# Autodesk Inventor assembly: GI - 100
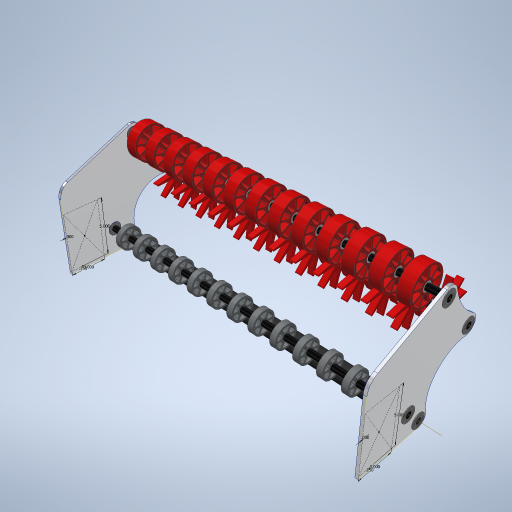
[picture p0: Inventor's stored thumbnail of the model, 512x512]
Saved by Autodesk Inventor 2023.4 (Build 274418000, 418)
## iProperties
Created: 2025-01-18
Part Number: GI - 100
Document SubType Name: Assembly
Designer: mavericks
Author: mavericks
## Documents named in this file (8)
- C:\Users\mavericks\Documents\GitHub\2025-ReefScape---CAD\ground intake\GI - 100.iam
- C:\Users\mavericks\Documents\GitHub\2025-ReefScape---CAD\ground intake\GI - 001.ipt
- C:\Users\mavericks\Documents\GitHub\2025-ReefScape---CAD\COMMON PARTS\BEARINGS\13_75mm_1_2_ThunderHex_ID_x_1_125_OD_x_0_313_WD_Flanged_Bearing_217-4006_MIR.ipt
- C:\Users\mavericks\Documents\GitHub\2025-ReefScape---CAD\ground intake\GI - 002.ipt
- C:\Users\mavericks\Documents\GitHub\2025-ReefScape---CAD\COMMON PARTS\WHEELS\am-0619a .425 Hex Entrapption Star REV2.ipt
- C:\Users\mavericks\Documents\GitHub\2025-ReefScape---CAD\COMMON PARTS\WHEELS\am-3946 3IN 375Hex Compliant Wheel REV 3.ipt
- C:\Users\mavericks\Documents\GitHub\2025-ReefScape---CAD\COMMON PARTS\WHEELS\2_OD_Straight_Flex_Wheel_217-6354.ipt
- C:\Users\mavericks\Documents\GitHub\2025-ReefScape---CAD\ground intake\GI - 200.iam
## Components (53 placed, 7 different names)
1. GI - 001:1 — Insert:1, Insert:2, Insert:3, Insert:4, Mate:2, Mate:4, Mate:6
2. 13_75mm_1_2_ThunderHex_ID_x_1_125_OD_x_0_313_WD_Flanged_Bearing_217-4006_MIR:1 — Insert:2, Insert:11, Mate:1
3. 13_75mm_1_2_ThunderHex_ID_x_1_125_OD_x_0_313_WD_Flanged_Bearing_217-4006_MIR:2 — Insert:1, Insert:12, Mate:3
4. 13_75mm_1_2_ThunderHex_ID_x_1_125_OD_x_0_313_WD_Flanged_Bearing_217-4006_MIR:3 — Insert:4, Insert:17
5. 13_75mm_1_2_ThunderHex_ID_x_1_125_OD_x_0_313_WD_Flanged_Bearing_217-4006_MIR:4 — Insert:3, Insert:10, Mate:5
6. GI - 001:2 — Insert:5, Insert:6, Insert:7, Insert:8
7. 13_75mm_1_2_ThunderHex_ID_x_1_125_OD_x_0_313_WD_Flanged_Bearing_217-4006_MIR:5 — Insert:5, Insert:13
8. 13_75mm_1_2_ThunderHex_ID_x_1_125_OD_x_0_313_WD_Flanged_Bearing_217-4006_MIR:6 — Insert:6, Insert:14
9. 13_75mm_1_2_ThunderHex_ID_x_1_125_OD_x_0_313_WD_Flanged_Bearing_217-4006_MIR:7 — Insert:8, Insert:16
10. 13_75mm_1_2_ThunderHex_ID_x_1_125_OD_x_0_313_WD_Flanged_Bearing_217-4006_MIR:8 — Insert:7, Insert:15
11. GI - 002:1 — Insert:12, Insert:14
12. GI - 002:2 — Insert:10, Insert:15
13. GI - 002:4 — Insert:11, Insert:13
14. GI - 200:1 [sub-assembly] — Insert:16, Insert:17
15. am-0619a .425 Hex Entrapption Star REV2:1 — Mate:1, Mate:2
16. am-0619a .425 Hex Entrapption Star REV2:2
17. am-0619a .425 Hex Entrapption Star REV2:3
18. am-0619a .425 Hex Entrapption Star REV2:4
19. am-0619a .425 Hex Entrapption Star REV2:5
20. am-0619a .425 Hex Entrapption Star REV2:6
21. am-0619a .425 Hex Entrapption Star REV2:7
22. am-0619a .425 Hex Entrapption Star REV2:8
23. am-0619a .425 Hex Entrapption Star REV2:9
24. am-0619a .425 Hex Entrapption Star REV2:10
25. am-0619a .425 Hex Entrapption Star REV2:11
26. am-0619a .425 Hex Entrapption Star REV2:12
27. am-0619a .425 Hex Entrapption Star REV2:13
28. am-3946 3IN 375Hex Compliant Wheel REV 3:1 — Mate:3, Mate:4
29. am-3946 3IN 375Hex Compliant Wheel REV 3:2
30. am-3946 3IN 375Hex Compliant Wheel REV 3:3
31. am-3946 3IN 375Hex Compliant Wheel REV 3:4
32. am-3946 3IN 375Hex Compliant Wheel REV 3:5
33. am-3946 3IN 375Hex Compliant Wheel REV 3:6
34. am-3946 3IN 375Hex Compliant Wheel REV 3:7
35. am-3946 3IN 375Hex Compliant Wheel REV 3:8
36. am-3946 3IN 375Hex Compliant Wheel REV 3:9
37. am-3946 3IN 375Hex Compliant Wheel REV 3:10
38. am-3946 3IN 375Hex Compliant Wheel REV 3:11
39. am-3946 3IN 375Hex Compliant Wheel REV 3:12
40. am-3946 3IN 375Hex Compliant Wheel REV 3:13
41. 2_OD_Straight_Flex_Wheel_217-6354:1 — Mate:5, Mate:6
42. 2_OD_Straight_Flex_Wheel_217-6354:2
43. 2_OD_Straight_Flex_Wheel_217-6354:3
44. 2_OD_Straight_Flex_Wheel_217-6354:4
45. 2_OD_Straight_Flex_Wheel_217-6354:5
46. 2_OD_Straight_Flex_Wheel_217-6354:6
47. 2_OD_Straight_Flex_Wheel_217-6354:7
48. 2_OD_Straight_Flex_Wheel_217-6354:8
49. 2_OD_Straight_Flex_Wheel_217-6354:9
50. 2_OD_Straight_Flex_Wheel_217-6354:10
51. 2_OD_Straight_Flex_Wheel_217-6354:11
52. 2_OD_Straight_Flex_Wheel_217-6354:12
53. 2_OD_Straight_Flex_Wheel_217-6354:13
## Component patterns: (13 elements, first: am-0619a .425 Hex Entrapption Star REV2:1), (13 elements, first: am-3946 3IN 375Hex Compliant Wheel REV 3:1), (13 elements, first: 2_OD_Straight_Flex_Wheel_217-6354:1)
## Relationships (22: Insert 16, Mate 6)
- Insert:1: GI - 001:1 ↔ 13_75mm_1_2_ThunderHex_ID_x_1_125_OD_x_0_313_WD_Flanged_Bearing_217-4006_MIR:2
- Insert:2: GI - 001:1 ↔ 13_75mm_1_2_ThunderHex_ID_x_1_125_OD_x_0_313_WD_Flanged_Bearing_217-4006_MIR:1
- Insert:3: GI - 001:1 ↔ 13_75mm_1_2_ThunderHex_ID_x_1_125_OD_x_0_313_WD_Flanged_Bearing_217-4006_MIR:4
- Insert:4: GI - 001:1 ↔ 13_75mm_1_2_ThunderHex_ID_x_1_125_OD_x_0_313_WD_Flanged_Bearing_217-4006_MIR:3
- Insert:5: GI - 001:2 ↔ 13_75mm_1_2_ThunderHex_ID_x_1_125_OD_x_0_313_WD_Flanged_Bearing_217-4006_MIR:5
- Insert:6: GI - 001:2 ↔ 13_75mm_1_2_ThunderHex_ID_x_1_125_OD_x_0_313_WD_Flanged_Bearing_217-4006_MIR:6
- Insert:7: GI - 001:2 ↔ 13_75mm_1_2_ThunderHex_ID_x_1_125_OD_x_0_313_WD_Flanged_Bearing_217-4006_MIR:8
- Insert:8: GI - 001:2 ↔ 13_75mm_1_2_ThunderHex_ID_x_1_125_OD_x_0_313_WD_Flanged_Bearing_217-4006_MIR:7
- Insert:10: 13_75mm_1_2_ThunderHex_ID_x_1_125_OD_x_0_313_WD_Flanged_Bearing_217-4006_MIR:4 ↔ GI - 002:2
- Insert:11: 13_75mm_1_2_ThunderHex_ID_x_1_125_OD_x_0_313_WD_Flanged_Bearing_217-4006_MIR:1 ↔ GI - 002:4
- Insert:12: 13_75mm_1_2_ThunderHex_ID_x_1_125_OD_x_0_313_WD_Flanged_Bearing_217-4006_MIR:2 ↔ GI - 002:1
- Insert:13: 13_75mm_1_2_ThunderHex_ID_x_1_125_OD_x_0_313_WD_Flanged_Bearing_217-4006_MIR:5 ↔ GI - 002:4
- Insert:14: 13_75mm_1_2_ThunderHex_ID_x_1_125_OD_x_0_313_WD_Flanged_Bearing_217-4006_MIR:6 ↔ GI - 002:1
- Insert:15: 13_75mm_1_2_ThunderHex_ID_x_1_125_OD_x_0_313_WD_Flanged_Bearing_217-4006_MIR:8 ↔ GI - 002:2
- Mate:1: 13_75mm_1_2_ThunderHex_ID_x_1_125_OD_x_0_313_WD_Flanged_Bearing_217-4006_MIR:1 ↔ am-0619a .425 Hex Entrapption Star REV2:1
- Mate:2 (36.5125 mm): GI - 001:1 ↔ am-0619a .425 Hex Entrapption Star REV2:1
- Mate:3: 13_75mm_1_2_ThunderHex_ID_x_1_125_OD_x_0_313_WD_Flanged_Bearing_217-4006_MIR:2 ↔ am-3946 3IN 375Hex Compliant Wheel REV 3:1
- Mate:4 (30.1625 mm): GI - 001:1 ↔ am-3946 3IN 375Hex Compliant Wheel REV 3:1
- Mate:5: 13_75mm_1_2_ThunderHex_ID_x_1_125_OD_x_0_313_WD_Flanged_Bearing_217-4006_MIR:4 ↔ 2_OD_Straight_Flex_Wheel_217-6354:1
- Mate:6 (36.5125 mm): GI - 001:1 ↔ 2_OD_Straight_Flex_Wheel_217-6354:1
- Insert:16: 13_75mm_1_2_ThunderHex_ID_x_1_125_OD_x_0_313_WD_Flanged_Bearing_217-4006_MIR:7 ↔ GI - 200:1
- Insert:17: 13_75mm_1_2_ThunderHex_ID_x_1_125_OD_x_0_313_WD_Flanged_Bearing_217-4006_MIR:3 ↔ GI - 200:1
